# Autodesk Inventor assembly: Lift Assembly Right
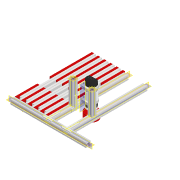
[picture p0: Inventor's stored thumbnail of the model, 180x180]
Saved by Autodesk Inventor 2020 (Build 240168000, 168)
## iProperties
Created: 2019-12-26
Part Number: Lift Assembly Right
Document SubType Name: Assembly
Designer: ball
Author: ball
## Documents named in this file (8)
- C:\FTC\FTC8863CAD\2019 Robot\Delivery\Lift Right\Lift Assembly Right.iam
- C:\FTC\FTC8863CAD\2019 Robot\Delivery\Lift Right\SAR330  x 5 + couplers right.iam
- C:\FTC\FTC8863CAD\Actobotics\565 parts\565046.ipt
- C:\FTC\FTC8863CAD\Actobotics\585 parts\585075.ipt
- C:\FTC\FTC8863CAD\Actobotics\565 parts\xrail_3.5in.ipt
- C:\FTC\FTC8863CAD\Actobotics\555 parts\555116 assembly.ipt
- C:\FTC\FTC8863CAD\Andymark\am-3461a NeveRest 4 with Motor REV3.ipt
- C:\FTC\FTC8863CAD\2019 Robot\Delivery\spool double 2 in diameter.iam
## Components (14 placed, 7 different names)
1. SAR330  x 5 + couplers right:1 [sub-assembly] — Mate:8, Flush:2, Flush:3, Mate:9, Flush:4, Flush:5, Mate:18, Mate:25, Mate:26
2. 565046:1 — Mate:8, Flush:2, Flush:3, Mate:10, Mate:11, Mate:12, Mate:13, Mate:14, Flush:7
3. 585075:2
4. 565046:2 — Mate:11, Mate:12, Flush:5, Flush:6, Mate:16, Mate:24, Flush:9
5. 585075:4 — Mate:9, Mate:10, Flush:4
6. xrail_3.5in:2 — Mate:16, Flush:7, Flush:8, Mate:24, Mate:28, Mate:29, Flush:12, Symmetry:1
7. 585075:5 — Mate:19, Mate:26, Mate:27
8. 585075:6 — Mate:13, Mate:14, Flush:6
9. xrail_3.5in:3 — Mate:18, Flush:8, Mate:19, Mate:25, Mate:27, Symmetry:1
10. 585075:8 — Flush:9, Mate:28, Mate:29
11. 555116 assembly:1 — Mate:34, Flush:10
12. 555116 assembly:2 — Mate:33, Flush:11
13. am-3461a NeveRest 4 with Motor REV3:1 — Mate:33, Mate:34, Flush:10, Flush:11, Flush:12, Mate:35, Mate:38, Mate:39
14. spool double 2 in diameter:1 [sub-assembly] — Mate:38, Mate:39
## Relationships (35: Mate 23, Flush 11, Symmetry 1)
- [Mate]: 565046:1 ↔ 585075:2
- [Mate]: 565046:1 ↔ 585075:2
- Mate:8: SAR330  x 5 + couplers right:1 ↔ 565046:1
- Flush:2: SAR330  x 5 + couplers right:1 ↔ 565046:1
- Flush:3: SAR330  x 5 + couplers right:1 ↔ 565046:1
- Mate:9: SAR330  x 5 + couplers right:1 ↔ 585075:4
- Mate:10: 565046:1 ↔ 585075:4
- Flush:4: SAR330  x 5 + couplers right:1 ↔ 585075:4
- Mate:11: 565046:1 ↔ 565046:2
- Mate:12: 565046:1 ↔ 565046:2
- Flush:5 (76.2 mm): SAR330  x 5 + couplers right:1 ↔ 565046:2
- Mate:13: 565046:1 ↔ 585075:6
- Mate:14: 565046:1 ↔ 585075:6
- Flush:6: 565046:2 ↔ 585075:6
- Mate:16: 565046:2 ↔ xrail_3.5in:2
- Flush:7 (-100.2792 mm): 565046:1 ↔ xrail_3.5in:2
- Mate:18: SAR330  x 5 + couplers right:1 ↔ xrail_3.5in:3
- Flush:8: xrail_3.5in:2 ↔ xrail_3.5in:3
- Mate:19: 585075:5 ↔ xrail_3.5in:3
- Mate:24: 565046:2 ↔ xrail_3.5in:2
- Mate:25: SAR330  x 5 + couplers right:1 ↔ xrail_3.5in:3
- Mate:26: SAR330  x 5 + couplers right:1 ↔ 585075:5
- Mate:27: 585075:5 ↔ xrail_3.5in:3
- Flush:9: 565046:2 ↔ 585075:8
- Mate:28: xrail_3.5in:2 ↔ 585075:8
- Mate:29: xrail_3.5in:2 ↔ 585075:8
- Mate:33: 555116 assembly:2 ↔ am-3461a NeveRest 4 with Motor REV3:1
- Mate:34: 555116 assembly:1 ↔ am-3461a NeveRest 4 with Motor REV3:1
- Flush:10 (22.86 mm): 555116 assembly:1 ↔ am-3461a NeveRest 4 with Motor REV3:1
- Flush:11 (19.05 mm): 555116 assembly:2 ↔ am-3461a NeveRest 4 with Motor REV3:1
- Flush:12: xrail_3.5in:2 ↔ am-3461a NeveRest 4 with Motor REV3:1
- Symmetry:1: xrail_3.5in:2 ↔ xrail_3.5in:3
- Mate:35: am-3461a NeveRest 4 with Motor REV3:1
- Mate:38: am-3461a NeveRest 4 with Motor REV3:1 ↔ spool double 2 in diameter:1
- Mate:39: am-3461a NeveRest 4 with Motor REV3:1 ↔ spool double 2 in diameter:1
